# Autodesk Inventor assembly: 3_stageGEM
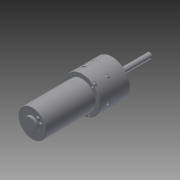
[picture p0: Inventor's stored thumbnail of the model, 180x180]
Saved by Autodesk Inventor 2015 (Build 190159000, 159)
## iProperties
Created: 2015-02-08
Part Number: 3_stageGEM
Document SubType Name: Assembly
Designer: pltwe4
Title: 3 stage GEM.STEP
Description: STEP AP203
Creation Date: 2010-07-19
Sending System: SolidWorks 2010
Preprocessor: SwSTEP 2.0
Author: pltwe4
## Documents named in this file (8)
- C:\Users\pltwe4\Documents\recycling-rush\model\3_stageGEM.iam
- C:\Users\pltwe4\Documents\recycling-rush\model\Imported Components\3_stageGEM\10-32 X -75 SHCS-1.ipt
- C:\Users\pltwe4\Documents\recycling-rush\model\Imported Components\3_stageGEM\Output Block-1.iam
- C:\Users\pltwe4\Documents\recycling-rush\model\Imported Components\3_stageGEM\2mm x 6 key.ipt
- C:\Users\pltwe4\Documents\recycling-rush\model\Imported Components\3_stageGEM\Stage-1.iam
- C:\Users\pltwe4\Documents\recycling-rush\model\Imported Components\3_stageGEM\CIM Mount-1.ipt
- C:\Users\pltwe4\Documents\recycling-rush\model\Imported Components\3_stageGEM\SUN Gear15-2_Inch - Spur gear 20DP 15T 14.5PA 0.375FW ---S15N3.0H2.0L0.3125N.ipt
- C:\Users\pltwe4\Documents\recycling-rush\model\Imported Components\CIMple Box\CIM motor.ipt
## Components (15 placed, 15 different names)
1. 10-32 X -75 SHCS-1_1
2. Output Block-1_2 [sub-assembly] — Mate:4, Mate:5
3. 10-32 X -75 SHCS-1_3
4. 2mm x 6 key_4
5. 10-32 X -75 SHCS-1_5 — Mate:2
6. 10-32 X -75 SHCS-1_6
7. 10-32 X -75 SHCS-1_7
8. Stage-1_8 [sub-assembly]
9. 10-32 X -75 SHCS-1_9
10. 10-32 X -75 SHCS-1_10
11. 10-32 X -75 SHCS-1_11
12. CIM Mount-1_12 — Mate:1, Mate:3
13. SUN Gear15-2_Inch - Spur gear 20DP 15T 14.5PA 0.375FW ---S15N3.0H2.0L0.3125N_13
14. Stage-1_14 [sub-assembly]
15. CIM motor:1 — Mate:1, Mate:2, Mate:3
## Relationships (5: Mate 5)
- Mate:1: CIM Mount-1_12 ↔ CIM motor:1
- Mate:2: 10-32 X -75 SHCS-1_5 ↔ CIM motor:1
- Mate:3: CIM Mount-1_12 ↔ CIM motor:1
- Mate:4: Output Block-1_2
- Mate:5: Output Block-1_2
